# Autodesk Inventor assembly: EL2-.200
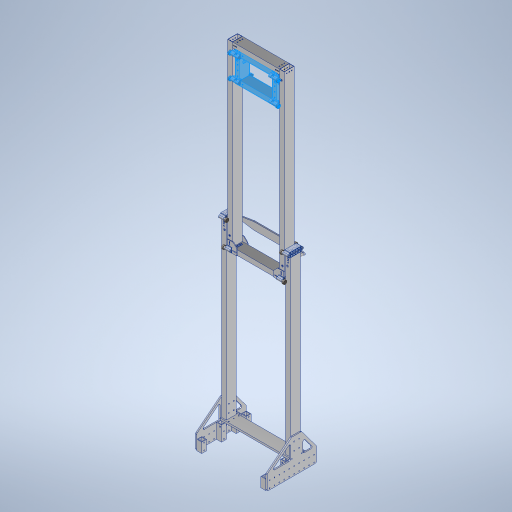
[picture p0: Inventor's stored thumbnail of the model, 512x512]
Saved by Autodesk Inventor 2023.4 (Build 274418000, 418)
## iProperties
Created: 2025-01-11
Part Number: EL2-.200
Document SubType Name: Assembly
Designer: slick
Author: slick
## Documents named in this file (11)
- C:\Users\mavericks\Desktop\2025-ReefScape---CAD\Elevator\EL2\EL2-.200.iam
- C:\Users\mavericks\Desktop\2025-ReefScape---CAD\Elevator\EL2\EL2-003.ipt
- C:\Users\mavericks\Desktop\2025-ReefScape---CAD\Elevator\EL2\EL2-.100.iam
- C:\Users\mavericks\Desktop\2025-ReefScape---CAD\Elevator\EL2\EL2-.300.iam
- C:\Users\mavericks\Desktop\2025-ReefScape---CAD\Elevator\EL2\EL2-C-100.iam
- C:\Users\mavericks\Desktop\2025-ReefScape---CAD\Elevator\EL2\EL2-012.ipt
- C:\Users\mavericks\Desktop\2025-ReefScape---CAD\Elevator\EL2\EL2-013.ipt
- C:\Users\mavericks\Desktop\2025-ReefScape---CAD\Elevator\EL2\EL2-S-002.ipt
- C:\Users\mavericks\Desktop\2025-ReefScape---CAD\Elevator\EL2\EL2-S-003.ipt
- C:\Users\mavericks\Desktop\2025-ReefScape---CAD\Elevator\EL2\EL2-S-004.ipt
- C:\Users\mavericks\Desktop\2025-ReefScape---CAD\Elevator\EL2\EL2-400A.iam
## Components (20 placed, 10 different names)
1. EL2-003:1 — Mate:3, Mate:7, Mate:8, Mate:9, Mate:10
2. EL2-.100:1 [sub-assembly] — Symmetry:1, Mate:2, Insert:10, Insert:19, Insert:22, Mate:10, Mate:11
3. EL2-.100:2 [sub-assembly] — Symmetry:1, Insert:9, Insert:20, Insert:21, Mate:8, Mate:9, Mate:13
4. EL2-.300:1 [sub-assembly] — Mate:1, Mate:2, Mate:3, Mate:4, Mate:15, Mate:16
5. EL2-C-100:1 [sub-assembly] — Mate:4, Mate:15, Mate:16
6. EL2-012:1 — Insert:7, Insert:9
7. EL2-012:2 — Insert:8, Insert:10
8. EL2-013:1 — Insert:7, Insert:8
9. EL2-S-002:1 — Insert:20, Insert:21, Mate:7, Insert:25, Insert:26, Insert:29, Insert:30, Insert:35, Insert:36, Insert:37, Insert:38
10. EL2-S-002:2 — Insert:19, Insert:22, Insert:23, Insert:24, Insert:27, Insert:28, Insert:31, Insert:32, Insert:33, Insert:34
11. EL2-S-003:1 — Insert:25, Insert:26
12. EL2-S-003:2 — Insert:23, Insert:24
13. EL2-S-003:3 — Insert:29, Insert:30
14. EL2-S-003:4 — Insert:27, Insert:28
15. EL2-S-004:1 — Insert:33, Insert:34, Mate:12
16. EL2-S-004:2 — Insert:31, Insert:32
17. EL2-S-004:3 — Insert:35, Insert:36, Mate:14
18. EL2-S-004:4 — Insert:37, Insert:38
19. EL2-400A:1 [sub-assembly] — Mate:11, Mate:12
20. EL2-400A:2 [sub-assembly] — Mate:13, Mate:14
## Relationships (39: Insert 24, Mate 14, Symmetry 1)
- Symmetry:1: EL2-.100:1 ↔ EL2-.100:2
- Mate:1: EL2-.300:1
- Mate:2: EL2-.100:1 ↔ EL2-.300:1
- Mate:3: EL2-003:1 ↔ EL2-.300:1
- Mate:4: EL2-.300:1 ↔ EL2-C-100:1
- Insert:7: EL2-012:1 ↔ EL2-013:1
- Insert:8: EL2-012:2 ↔ EL2-013:1
- Insert:9: EL2-.100:2 ↔ EL2-012:1
- Insert:10: EL2-.100:1 ↔ EL2-012:2
- Insert:19: EL2-.100:1 ↔ EL2-S-002:2
- Insert:20: EL2-.100:2 ↔ EL2-S-002:1
- Insert:21: EL2-.100:2 ↔ EL2-S-002:1
- Insert:22: EL2-.100:1 ↔ EL2-S-002:2
- Mate:7: EL2-003:1 ↔ EL2-S-002:1
- Mate:8: EL2-003:1 ↔ EL2-.100:2
- Mate:9: EL2-003:1 ↔ EL2-.100:2
- Mate:10: EL2-003:1 ↔ EL2-.100:1
- Insert:23: EL2-S-002:2 ↔ EL2-S-003:2
- Insert:24: EL2-S-002:2 ↔ EL2-S-003:2
- Insert:25: EL2-S-002:1 ↔ EL2-S-003:1
- Insert:26: EL2-S-002:1 ↔ EL2-S-003:1
- Insert:27: EL2-S-002:2 ↔ EL2-S-003:4
- Insert:28: EL2-S-002:2 ↔ EL2-S-003:4
- Insert:29: EL2-S-002:1 ↔ EL2-S-003:3
- Insert:30: EL2-S-002:1 ↔ EL2-S-003:3
- Insert:31: EL2-S-002:2 ↔ EL2-S-004:2
- Insert:32: EL2-S-002:2 ↔ EL2-S-004:2
- Insert:33: EL2-S-002:2 ↔ EL2-S-004:1
- Insert:34: EL2-S-002:2 ↔ EL2-S-004:1
- Insert:35: EL2-S-002:1 ↔ EL2-S-004:3
- Insert:36: EL2-S-002:1 ↔ EL2-S-004:3
- Mate:11: EL2-.100:1 ↔ EL2-400A:1
- Mate:12: EL2-S-004:1 ↔ EL2-400A:1
- Mate:13: EL2-.100:2 ↔ EL2-400A:2
- Mate:14: EL2-S-004:3 ↔ EL2-400A:2
- Insert:37: EL2-S-002:1 ↔ EL2-S-004:4
- Insert:38: EL2-S-002:1 ↔ EL2-S-004:4
- Mate:15: EL2-.300:1 ↔ EL2-C-100:1
- Mate:16: EL2-.300:1 ↔ EL2-C-100:1
